# Autodesk Inventor assembly: Hybrid
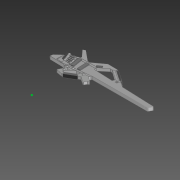
[picture p0: Inventor's stored thumbnail of the model, 180x180]
Saved by Autodesk Inventor 2020 (Build 240168000, 168)
## iProperties
Created: 2022-11-11
Part Number: Hybrid
Document SubType Name: Assembly
Designer: valer
Author: valer
## Documents named in this file (8)
- C:\Users\valer\Desktop\hybrid\src\Hybrid.iam
- C:\Users\valer\Desktop\hybrid\src\Hybrid.ipt
- C:\Users\valer\Desktop\hybrid\src\01BinaryLogo.ipt
- C:\Users\valer\Desktop\hybrid\src\OscilloscopeScreen.ipt
- C:\Users\valer\Desktop\hybrid\src\BottomGrip.ipt
- C:\Users\valer\Desktop\hybrid\src\TopGrip.ipt
- C:\Users\valer\Desktop\hybrid\src\BassTuner.ipt
- C:\Users\valer\Desktop\hybrid\src\MidiPickup.ipt
## Components (11 placed, 7 different names)
1. Hybrid:1 — Flush:2, Mate:2, Mate:3, Mate:4, Mate:5, Mate:6, Mate:13, Mate:14, Mate:15
2. 01BinaryLogo:1 — Mate:4, Mate:5, Mate:6
3. OscilloscopeScreen:1 — Flush:2, Mate:2, Mate:3
4. BottomGrip:1 — Mate:14, Mate:15
5. TopGrip:1
6. BassTuner:1
7. BassTuner:2
8. BassTuner:3
9. BassTuner:4
10. BassTuner:5
11. MidiPickup:1 — Mate:13
## Relationships (9: Mate 8, Flush 1)
- Flush:2: Hybrid:1 ↔ OscilloscopeScreen:1
- Mate:2: Hybrid:1 ↔ OscilloscopeScreen:1
- Mate:3: Hybrid:1 ↔ OscilloscopeScreen:1
- Mate:4: Hybrid:1 ↔ 01BinaryLogo:1
- Mate:5: Hybrid:1 ↔ 01BinaryLogo:1
- Mate:6: Hybrid:1 ↔ 01BinaryLogo:1
- Mate:13: Hybrid:1 ↔ MidiPickup:1
- Mate:14: Hybrid:1 ↔ BottomGrip:1
- Mate:15: Hybrid:1 ↔ BottomGrip:1
